# Autodesk Inventor assembly: ShaftCoupler
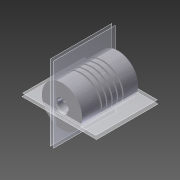
[picture p0: Inventor's stored thumbnail of the model, 180x180]
Saved by Autodesk Inventor 2015 (Build 190159000, 159)
## iProperties
Created: 2014-07-10
Part Number: ShaftCoupler
Document SubType Name: Assembly
Designer: t_clevj
Author: t_clevj
## Documents named in this file (3)
- C:\Users\t_clevj\Dropbox\Projects\AdamProjects\LinearActuator\ShaftCoupler\ShaftCoupler.iam
- C:\Users\t_clevj\Dropbox\Projects\AdamProjects\LinearActuator\ShaftCoupler\ShaftCouplerBody.ipt
- C:\Users\t_clevj\Dropbox\Projects\AdamProjects\LibHardware\Bolts\SetScrews\SetScrew3.ipt
## Components (5 placed, 2 different names)
1. ShaftCouplerBody:1 — Mate:1, Mate:2, Mate:3, Mate:4, Mate:5, Tangent:1, Tangent:2
2. SetScrew3:1 — Mate:2, Flush:7
3. SetScrew3:2 — Mate:3, Flush:2
4. SetScrew3:3 — Mate:1, Flush:6
5. SetScrew3:4 — Mate:4, Flush:8
## Relationships (15: Flush 8, Mate 5, Tangent 2)
- Mate:1: ShaftCouplerBody:1 ↔ SetScrew3:3
- Mate:2: ShaftCouplerBody:1 ↔ SetScrew3:1
- Mate:3: ShaftCouplerBody:1 ↔ SetScrew3:2
- Mate:4: ShaftCouplerBody:1 ↔ SetScrew3:4
- Mate:5: ShaftCouplerBody:1
- Tangent:1: ShaftCouplerBody:1
- Tangent:2: ShaftCouplerBody:1
- Flush:1 (5 mm)
- Flush:2: SetScrew3:2
- Flush:3 (-13 mm)
- Flush:4 (6.5 mm)
- Flush:5 (-11.5 mm)
- Flush:6: SetScrew3:3
- Flush:7: SetScrew3:1
- Flush:8: SetScrew3:4
